# Autodesk Inventor assembly: assem_palm_test_v1
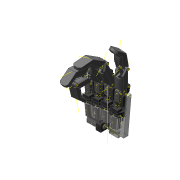
[picture p0: Inventor's stored thumbnail of the model, 180x180]
Saved by Autodesk Inventor 2014 (Build 180170000, 170)
## iProperties
Created: 2015-05-07
Part Number: assem_palm_test_v1
Document SubType Name: Assembly
Designer: Martin
Author: Martin
## Documents named in this file (11)
- C:\Users\Martin\Dropbox\biohand-mec\biohand_v1\palm\assem_palm_test_v1.iam
- C:\Users\Martin\Dropbox\biohand-mec\biohand_v1\fingers\index\assem_finger_index.iam
- C:\Users\Martin\Dropbox\biohand-mec\biohand_v1\fingers\middle\assem_finger_middle.iam
- C:\Users\Martin\Dropbox\biohand-mec\biohand_v1\fingers\ring\assem_finger_ring.iam
- C:\Users\Martin\Dropbox\biohand-mec\biohand_v1\fingers\pinky\assem_finger_pinky.iam
- C:\Users\Martin\Dropbox\biohand-mec\biohand_v1\misc\servo_square_pot.ipt
- C:\Users\Martin\Dropbox\biohand-mec\biohand_v1\palm\assem_palm_linact_v2.iam
- C:\Users\Martin\Dropbox\biohand-mec\biohand_v1\palm\palm_back_v3.ipt
- C:\Users\Martin\Dropbox\biohand-mec\biohand_v1\palm\linact_palm_rod.ipt
- C:\Users\Martin\Dropbox\biohand-mec\biohand_v1\misc\m3_nut.ipt
- C:\Users\Martin\Dropbox\biohand-mec\biohand_v1\misc\m2_8_screw.ipt
## Components (11 placed, 10 different names)
1. palm_back_v3:1 — Flush:1, Flush:2, Flush:3, Mate:1, Mate:2, Mate:3, Mate:4, Mate:5, Mate:6, Mate:7, Mate:8, Mate:9, Mate:10, Mate:11, Mate:12, Mate:13, Mate:14, Mate:15, Angle:1, Angle:2
2. assem_finger_index:1 [sub-assembly] — Mate:1, Mate:2, Mate:3
3. assem_finger_middle:1 [sub-assembly] — Mate:4, Mate:7, Mate:10
4. assem_finger_ring:1 [sub-assembly] — Mate:5, Mate:8, Mate:11
5. assem_finger_pinky:1 [sub-assembly] — Mate:6, Mate:9, Mate:12
6. servo_square_pot:1 — Angle:2, Angle:3
7. assem_palm_linact_v2:1 [sub-assembly] — Mate:13, Mate:14, Mate:15, Mate:17
8. linact_palm_rod:1 — Mate:17, Angle:1, Insert:1, Insert:2, Insert:3
9. m3_nut:1 — Insert:1
10. m2_8_screw:1 — Insert:3
11. m2_8_screw:2 — Insert:2
## Relationships (25: Mate 16, Flush 3, Angle 3, Insert 3)
- Flush:1: palm_back_v3:1
- Flush:2: palm_back_v3:1
- Flush:3: palm_back_v3:1
- Mate:1: palm_back_v3:1 ↔ assem_finger_index:1
- Mate:2: palm_back_v3:1 ↔ assem_finger_index:1
- Mate:3: palm_back_v3:1 ↔ assem_finger_index:1
- Mate:4: palm_back_v3:1 ↔ assem_finger_middle:1
- Mate:5: palm_back_v3:1 ↔ assem_finger_ring:1
- Mate:6: palm_back_v3:1 ↔ assem_finger_pinky:1
- Mate:7: palm_back_v3:1 ↔ assem_finger_middle:1
- Mate:8: palm_back_v3:1 ↔ assem_finger_ring:1
- Mate:9: palm_back_v3:1 ↔ assem_finger_pinky:1
- Mate:10: palm_back_v3:1 ↔ assem_finger_middle:1
- Mate:11: palm_back_v3:1 ↔ assem_finger_ring:1
- Mate:12: palm_back_v3:1 ↔ assem_finger_pinky:1
- Mate:13: palm_back_v3:1 ↔ assem_palm_linact_v2:1
- Mate:14: palm_back_v3:1 ↔ assem_palm_linact_v2:1
- Mate:15: palm_back_v3:1 ↔ assem_palm_linact_v2:1
- Mate:17: assem_palm_linact_v2:1 ↔ linact_palm_rod:1
- Angle:1 (180 deg): palm_back_v3:1 ↔ linact_palm_rod:1
- Insert:1: linact_palm_rod:1 ↔ m3_nut:1
- Insert:2: linact_palm_rod:1 ↔ m2_8_screw:2
- Insert:3: linact_palm_rod:1 ↔ m2_8_screw:1
- Angle:2 (0 deg): palm_back_v3:1 ↔ servo_square_pot:1
- Angle:3 (0 deg): servo_square_pot:1
